# Autodesk Inventor assembly: experimentAssembly
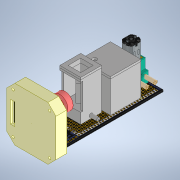
[picture p0: Inventor's stored thumbnail of the model, 180x180]
Saved by Autodesk Inventor 2020 (Build 240168000, 168)
## iProperties
Created: 2022-09-15
Part Number: experimentAssembly
Document SubType Name: Assembly
Designer: kouda
Author: kouda
## Documents named in this file (12)
- D:\IRL\2022-2023\cads\experimentAssembly.iam
- D:\IRL\2022-2023\cads\MicroLab_Center_Shell.ipt
- D:\IRL\2022-2023\cads\MicroLab_Rear_Cover.ipt
- D:\IRL\2022-2023\cads\MicroLab_PCB_002 (2).ipt
- D:\IRL\2022-2023\cads\C329-SPI.ipt
- D:\IRL\2022-2023\cads\latticeChamberv4.ipt
- D:\IRL\2022-2023\cads\latticeChamberCapv4.ipt
- D:\IRL\2022-2023\cads\latticeStandIn.ipt
- D:\IRL\2022-2023\cads\RapidProto2PCB_by_Lim.ipt
- D:\IRL\2022-2023\cads\waterBallonHolderCapv2.ipt
- D:\IRL\2022-2023\cads\waterBallonHolderv2.ipt
- D:\IRL\2022-2023\cads\MPP20-E20_by_Lim.ipt
## Components (11 placed, 11 different names)
1. MicroLab_Center_Shell:2 — Mate:1, Mate:2, Flush:1
2. MicroLab_Rear_Cover:1 — Mate:1, Mate:2, Flush:1, Mate:3, Mate:5, Mate:6
3. MicroLab_PCB_002 (2):1 — Mate:3, Mate:5, Mate:6, Mate:7, Mate:8, Mate:9, Mate:15, Flush:6, Mate:16
4. latticeChamberv4:1 — Mate:10, Flush:2, Flush:3, Mate:11, Mate:12, Mate:13, Mate:14, Flush:5, Flush:10
5. C329-SPI:1 — Mate:7, Mate:8, Mate:9, Mate:11, Flush:4, Flush:5
6. latticeChamberCapv4:1 — Mate:10, Flush:2, Flush:3
7. latticeStandIn:1 — Mate:12, Mate:13, Mate:14, Flush:4
8. RapidProto2PCB_by_Lim:1 — Mate:15, Flush:6, Mate:16, Flush:9
9. waterBallonHolderv2:1 — Mate:17, Flush:7, Flush:8, Flush:9, Flush:10, Mate:18, Flush:12
10. waterBallonHolderCapv2:1 — Mate:17, Flush:7, Flush:8, Flush:11
11. MPP20-E20_by_Lim:1 — Flush:11, Mate:18, Flush:12
## Relationships (29: Mate 17, Flush 12)
- Mate:1: MicroLab_Center_Shell:2 ↔ MicroLab_Rear_Cover:1
- Mate:2: MicroLab_Center_Shell:2 ↔ MicroLab_Rear_Cover:1
- Flush:1: MicroLab_Center_Shell:2 ↔ MicroLab_Rear_Cover:1
- Mate:3: MicroLab_Rear_Cover:1 ↔ MicroLab_PCB_002 (2):1
- Mate:5: MicroLab_Rear_Cover:1 ↔ MicroLab_PCB_002 (2):1
- Mate:6: MicroLab_Rear_Cover:1 ↔ MicroLab_PCB_002 (2):1
- Mate:7: MicroLab_PCB_002 (2):1 ↔ C329-SPI:1
- Mate:8: MicroLab_PCB_002 (2):1 ↔ C329-SPI:1
- Mate:9: MicroLab_PCB_002 (2):1 ↔ C329-SPI:1
- Mate:10: latticeChamberv4:1 ↔ latticeChamberCapv4:1
- Flush:2: latticeChamberv4:1 ↔ latticeChamberCapv4:1
- Flush:3: latticeChamberv4:1 ↔ latticeChamberCapv4:1
- Mate:11 (7 mm): latticeChamberv4:1 ↔ C329-SPI:1
- Mate:12: latticeChamberv4:1 ↔ latticeStandIn:1
- Mate:13: latticeChamberv4:1 ↔ latticeStandIn:1
- Mate:14: latticeChamberv4:1 ↔ latticeStandIn:1
- Flush:4 (-2.25 mm): C329-SPI:1 ↔ latticeStandIn:1
- Flush:5 (-3 mm): latticeChamberv4:1 ↔ C329-SPI:1
- Mate:15: MicroLab_PCB_002 (2):1 ↔ RapidProto2PCB_by_Lim:1
- Flush:6 (-1.1215 mm): MicroLab_PCB_002 (2):1 ↔ RapidProto2PCB_by_Lim:1
- Mate:16: MicroLab_PCB_002 (2):1 ↔ RapidProto2PCB_by_Lim:1
- Mate:17: waterBallonHolderv2:1 ↔ waterBallonHolderCapv2:1
- Flush:7: waterBallonHolderv2:1 ↔ waterBallonHolderCapv2:1
- Flush:8: waterBallonHolderv2:1 ↔ waterBallonHolderCapv2:1
- Flush:9: RapidProto2PCB_by_Lim:1 ↔ waterBallonHolderv2:1
- Flush:10: latticeChamberv4:1 ↔ waterBallonHolderv2:1
- Flush:11: waterBallonHolderCapv2:1 ↔ MPP20-E20_by_Lim:1
- Mate:18 (5 mm): waterBallonHolderv2:1 ↔ MPP20-E20_by_Lim:1
- Flush:12: waterBallonHolderv2:1 ↔ MPP20-E20_by_Lim:1
